# Autodesk Inventor assembly: InitialAssembly
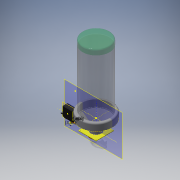
[picture p0: Inventor's stored thumbnail of the model, 180x180]
Saved by Autodesk Inventor 2019 (Build 230136000, 136)
## iProperties
Created: 2018-12-14
Part Number: InitialAssembly
Document SubType Name: Assembly
Designer: assman
Author: assman
## Documents named in this file (9)
- D:\Inventor\Projects\CatFeeder\Initial Version\InitialAssembly.iam
- D:\Inventor\Projects\CatFeeder\Initial Version\Jar.ipt
- D:\Inventor\Projects\CatFeeder\Initial Version\ServoDock.ipt
- D:\Inventor\Projects\3party\Servos\MG995.ipt
- D:\Inventor\Projects\CatFeeder\Initial Version\JarCone.ipt
- D:\Inventor\Projects\CatFeeder\Initial Version\TrapAdapter.ipt
- D:\Inventor\Projects\CatFeeder\Initial Version\Trap.ipt
- D:\Inventor\Projects\CatFeeder\Initial Version\TrapLimiter.ipt
- D:\Inventor\Projects\CatFeeder\Initial Version\LowerBox.ipt
## Components (8 placed, 8 different names)
1. Jar:1 — Rigid:1
2. ServoDock:1 — Rigid:2, Rigid:3, Rigid:4
3. JarCone:1 — Rigid:1, Rigid:2
4. MG995:1 — Rigid:3, Flush:1, Flush:2, Rotational:1
5. TrapAdapter:1 — Rigid:4
6. Trap:1 — Rotational:1, Flush:3, Flush:4, Rigid:5
7. TrapLimiter:1 — Flush:3, Flush:4, Rigid:5, Flush:10, Flush:11
8. LowerBox:1 — Flush:7, Flush:9, Flush:11
## Relationships (18: Flush 10, WeldJoint 5, Symmetry 2, RevoluteJoint 1)
- Rigid:1 [WeldJoint]: Jar:1 ↔ JarCone:1
- Rigid:2 [WeldJoint]: ServoDock:1 ↔ JarCone:1
- Rigid:3 [WeldJoint]: ServoDock:1 ↔ MG995:1
- Flush:1: MG995:1
- Flush:2: MG995:1
- Symmetry:1
- Rigid:4 [WeldJoint]: ServoDock:1 ↔ TrapAdapter:1
- Rotational:1 [RevoluteJoint]: MG995:1 ↔ Trap:1
- Flush:3: Trap:1 ↔ TrapLimiter:1
- Flush:4: Trap:1 ↔ TrapLimiter:1
- Rigid:5 [WeldJoint]: Trap:1 ↔ TrapLimiter:1
- Symmetry:2
- Flush:6
- Flush:7: LowerBox:1
- Flush:8 (-20 mm)
- Flush:9: LowerBox:1
- Flush:10 (5 mm): TrapLimiter:1
- Flush:11 (5 mm): TrapLimiter:1 ↔ LowerBox:1
